# Autodesk Inventor assembly: 742a 2.1 Catapult
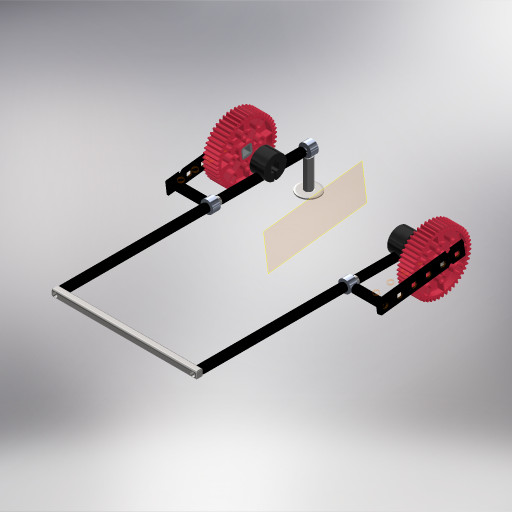
[picture p0: Inventor's stored thumbnail of the model, 512x512]
Saved by Autodesk Inventor 2024 (Build 280153000, 153)
## iProperties
Created: 2023-10-21
Part Number: 742a 2.1 Catapult
Document SubType Name: Assembly
Designer: aaron
Author: aaron
## Documents named in this file (12)
- C:\Users\aaron\Documents\Inventor\TritonRobotics\library\Subsystems\742a 2.1 Catapult.iam
- C:\Users\aaron\Documents\Inventor\TritonRobotics\library\VEX Library\Motion\HS Shaft\HS Shaft Collar.ipt
- C:\Users\aaron\Documents\Inventor\TritonRobotics\library\VEX Library\Structure\Standoff.ipt
- C:\Users\aaron\Documents\Inventor\TritonRobotics\library\VEX Library\Motion\Gears\High Strength\48 Tooth\48 High Strength Gear V2.ipt
- C:\Users\aaron\Documents\Inventor\TritonRobotics\library\VEX Library\Structure\C-Channels\Aluminum 1x1 from VEX\1x1x6 Aluminum Angle.ipt
- C:\Users\aaron\Documents\Inventor\TritonRobotics\library\VEX Library\Structure\Standoff\Standoff 1.5.ipt
- C:\Users\aaron\Documents\Inventor\TritonRobotics\library\VEX Library\Structure\Metal Spacers\.125 .25 OD.ipt
- C:\Users\aaron\Documents\Inventor\TritonRobotics\library\VEX Library\Motion\Shaft Collar with Set Screw.ipt
- C:\Users\aaron\Documents\Inventor\TritonRobotics\library\VEX Library\Structure\Standoff\Standoff 5.ipt
- C:\Users\aaron\Documents\Inventor\TritonRobotics\library\VEX Library\Structure\hs shaft\cata Beam.ipt
- C:\Users\aaron\Documents\Inventor\TritonRobotics\library\VEX Library\Structure\Standoff\Standoff 1.ipt
- C:\Users\aaron\Documents\Inventor\TritonRobotics\library\VEX Library\Motion\Spacers\0.75 od spcaer.ipt
## Components (25 placed, 10 different names)
1. HS Shaft Collar:1 — Mate:1, Mate:6, Mate:15, Mate:16, Mate:53, Mate:54
2. HS Shaft Collar:2 — Mate:1, Mate:7, Mate:14, Mate:17, Mate:55, Mate:56
3. 48 High Strength Gear V2:1 — Mate:6, Mate:8, Mate:9, Mate:10
4. 48 High Strength Gear V2:2 — Mate:7, Mate:11, Mate:12, Mate:13
5. 1x1x6 Aluminum Angle:1 — Mate:11, Mate:12, Mate:13, Mate:18, Mate:34, Symmetry:1, Mate:48, Mate:49
6. 1x1x6 Aluminum Angle:4 — Mate:8, Mate:9, Mate:10, Mate:18, Mate:28, Symmetry:1, Mate:50, Mate:51
7. Standoff 1.5:1 — Mate:15, Mate:16, Mate:25, Mate:26, Mate:27
8. Standoff 1.5:2 — Mate:14, Mate:17, Mate:23, Mate:24
9. .125 .25 OD:1 — Mate:25, Mate:26
10. .125 .25 OD:2 — Mate:23, Mate:24, Mate:33
11. Shaft Collar with Set Screw:1 — Mate:27, Mate:28, Mate:40, Mate:41, Mate:52
12. Shaft Collar with Set Screw:2 — Mate:33, Mate:34, Mate:39, Mate:42, Mate:46, Mate:47
13. Standoff 5:5 — Mate:39, Mate:42, Mate:43
14. Standoff 5:6 — Mate:40, Mate:41, Mate:44, Mate:45
15. cata Beam:1 — Mate:43, Mate:44, Mate:45
16. Standoff 1:7 — Mate:50, Mate:51, Mate:52
17. Standoff 1:8 — Mate:46, Mate:47, Mate:48, Mate:49
18. Standoff 1:9 — Mate:53, Mate:54, Mate:62, Mate:63
19. Standoff 1:10 — Mate:55, Mate:56, Mate:59
20. Shaft Collar with Set Screw:3 — Mate:59
21. Standoff 1:11 — Flush:1, Mate:65, Mate:66
22. Shaft Collar with Set Screw:4 — Mate:62, Mate:63
23. Standoff 1:12 — Flush:1, Mate:64, Mate:67
24. 0.75 od spcaer:1 — Mate:65, Mate:66
25. 0.75 od spcaer:2 — Mate:64, Mate:67
## Relationships (53: Mate 51, Symmetry 1, Flush 1)
- Mate:1: HS Shaft Collar:1 ↔ HS Shaft Collar:2
- Mate:6: HS Shaft Collar:1 ↔ 48 High Strength Gear V2:1
- Mate:7: HS Shaft Collar:2 ↔ 48 High Strength Gear V2:2
- Mate:8: 48 High Strength Gear V2:1 ↔ 1x1x6 Aluminum Angle:4
- Mate:9: 48 High Strength Gear V2:1 ↔ 1x1x6 Aluminum Angle:4
- Mate:10: 48 High Strength Gear V2:1 ↔ 1x1x6 Aluminum Angle:4
- Mate:11: 48 High Strength Gear V2:2 ↔ 1x1x6 Aluminum Angle:1
- Mate:12: 48 High Strength Gear V2:2 ↔ 1x1x6 Aluminum Angle:1
- Mate:13: 48 High Strength Gear V2:2 ↔ 1x1x6 Aluminum Angle:1
- Mate:14: HS Shaft Collar:2 ↔ Standoff 1.5:2
- Mate:15: HS Shaft Collar:1 ↔ Standoff 1.5:1
- Mate:16: HS Shaft Collar:1 ↔ Standoff 1.5:1
- Mate:17: HS Shaft Collar:2 ↔ Standoff 1.5:2
- Mate:18: 1x1x6 Aluminum Angle:1 ↔ 1x1x6 Aluminum Angle:4
- Mate:23: Standoff 1.5:2 ↔ .125 .25 OD:2
- Mate:24: Standoff 1.5:2 ↔ .125 .25 OD:2
- Mate:25: Standoff 1.5:1 ↔ .125 .25 OD:1
- Mate:26: Standoff 1.5:1 ↔ .125 .25 OD:1
- Mate:27: Standoff 1.5:1 ↔ Shaft Collar with Set Screw:1
- Mate:28: 1x1x6 Aluminum Angle:4 ↔ Shaft Collar with Set Screw:1
- Mate:33: .125 .25 OD:2 ↔ Shaft Collar with Set Screw:2
- Mate:34: 1x1x6 Aluminum Angle:1 ↔ Shaft Collar with Set Screw:2
- Mate:39: Shaft Collar with Set Screw:2 ↔ Standoff 5:5
- Mate:40: Shaft Collar with Set Screw:1 ↔ Standoff 5:6
- Mate:41: Shaft Collar with Set Screw:1 ↔ Standoff 5:6
- Mate:42: Shaft Collar with Set Screw:2 ↔ Standoff 5:5
- Mate:43: Standoff 5:5 ↔ cata Beam:1
- Mate:44: Standoff 5:6 ↔ cata Beam:1
- Mate:45: Standoff 5:6 ↔ cata Beam:1
- Symmetry:1: 1x1x6 Aluminum Angle:1 ↔ 1x1x6 Aluminum Angle:4
- Mate:46: Shaft Collar with Set Screw:2 ↔ Standoff 1:8
- Mate:47: Shaft Collar with Set Screw:2 ↔ Standoff 1:8
- Mate:48: 1x1x6 Aluminum Angle:1 ↔ Standoff 1:8
- Mate:49: 1x1x6 Aluminum Angle:1 ↔ Standoff 1:8
- Mate:50: 1x1x6 Aluminum Angle:4 ↔ Standoff 1:7
- Mate:51: 1x1x6 Aluminum Angle:4 ↔ Standoff 1:7
- Mate:52: Shaft Collar with Set Screw:1 ↔ Standoff 1:7
- Mate:53: HS Shaft Collar:1 ↔ Standoff 1:9
- Mate:54: HS Shaft Collar:1 ↔ Standoff 1:9
- Mate:55: HS Shaft Collar:2 ↔ Standoff 1:10
- Mate:56: HS Shaft Collar:2 ↔ Standoff 1:10
- [Mate]: Shaft Collar with Set Screw:3 ↔ Standoff 1:11
- [Mate]: Shaft Collar with Set Screw:3 ↔ Standoff 1:11
- Mate:59: Standoff 1:10 ↔ Shaft Collar with Set Screw:3
- [Mate]: Shaft Collar with Set Screw:4 ↔ Standoff 1:12
- [Mate]: Shaft Collar with Set Screw:4 ↔ Standoff 1:12
- Mate:62: Standoff 1:9 ↔ Shaft Collar with Set Screw:4
- Mate:63: Standoff 1:9 ↔ Shaft Collar with Set Screw:4
- Flush:1: Standoff 1:11 ↔ Standoff 1:12
- Mate:64: Standoff 1:12 ↔ 0.75 od spcaer:2
- Mate:65: Standoff 1:11 ↔ 0.75 od spcaer:1
- Mate:66: Standoff 1:11 ↔ 0.75 od spcaer:1
- Mate:67: Standoff 1:12 ↔ 0.75 od spcaer:2
## Named parameters: d66_d51 = 0 mm, d67_d52 = 0 mm, d69_d51 = 0 mm, d70_d52 = 0 mm
